# Autodesk Inventor assembly: RightGantryMount
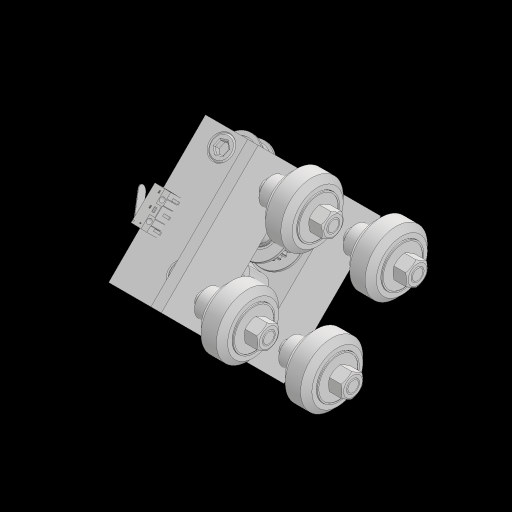
[picture p0: Inventor's stored thumbnail of the model, 512x512]
Saved by Autodesk Inventor 2023 (Build 270158000, 158)
## iProperties
Created: 2023-07-18
Part Number: RightGantryMount
Document SubType Name: Assembly
Designer: tandu
Author: tandu
## Documents named in this file (8)
- C:\Users\tandu\Documents\GrabCAD\Custom Conveyor Belt 3D Printer\References\Roller based conveyor belt 3d printer\RightGantryMount.iam
- C:\Users\tandu\Documents\GrabCAD\Custom Conveyor Belt 3D Printer\References\Roller based conveyor belt 3d printer\RollerVersiongantry_mount_right_bottom_v2.ipt
- C:\Users\tandu\Documents\GrabCAD\Custom Conveyor Belt 3D Printer\References\Roller based conveyor belt 3d printer\RollerVersionGates_2GT_20T_Toothed_Idler_Vychoz¡.ipt
- C:\Users\tandu\Documents\GrabCAD\Custom Conveyor Belt 3D Printer\References\Roller based conveyor belt 3d printer\RollerVersionF695 Bearing.step.ipt
- C:\Users\tandu\Documents\GrabCAD\Custom Conveyor Belt 3D Printer\References\Roller based conveyor belt 3d printer\RollerVersiongantry_mount_right_top_v2.ipt
- C:\Users\tandu\Documents\GrabCAD\Custom Conveyor Belt 3D Printer\References\Roller based conveyor belt 3d printer\RollerVersionM5x40.ipt
- C:\Users\tandu\Documents\GrabCAD\Custom Conveyor Belt 3D Printer\References\Roller based conveyor belt 3d printer\RollerVersionMicroswitch2.step.iam
- C:\Users\tandu\Documents\GrabCAD\Custom Conveyor Belt 3D Printer\References\Roller based conveyor belt 3d printer\RollerVersionSVWB.iam
## Components (13 placed, 7 different names)
1. RollerVersiongantry_mount_right_bottom_v2:1 — Insert:3, Insert:4, Insert:8, Mate:1
2. RollerVersionGates_2GT_20T_Toothed_Idler_Vychoz¡:1 — Insert:7
3. RollerVersionF695 Bearing.step:1 — Insert:6
4. RollerVersionF695 Bearing.step:2 — Insert:5, Insert:6
5. RollerVersiongantry_mount_right_top_v2:1 — Insert:1, Insert:2, Insert:5, Insert:7, Insert:8, Mate:1, Insert:9, Insert:10, Insert:11
6. RollerVersionM5x40:1 — Insert:10
7. RollerVersionM5x40:2 — Insert:9
8. RollerVersionM5x40:3 — Insert:11
9. RollerVersionMicroswitch2.step:1 [sub-assembly]
10. RollerVersionSVWB:1 [sub-assembly] — Insert:2
11. RollerVersionSVWB:2 [sub-assembly] — Insert:4
12. RollerVersionSVWB:3 [sub-assembly] — Insert:3
13. RollerVersionSVWB:4 [sub-assembly] — Insert:1
## Relationships (12: Insert 11, Mate 1)
- Insert:1: RollerVersiongantry_mount_right_top_v2:1 ↔ RollerVersionSVWB:4
- Insert:2: RollerVersiongantry_mount_right_top_v2:1 ↔ RollerVersionSVWB:1
- Insert:3: RollerVersiongantry_mount_right_bottom_v2:1 ↔ RollerVersionSVWB:3
- Insert:4: RollerVersiongantry_mount_right_bottom_v2:1 ↔ RollerVersionSVWB:2
- Insert:5: RollerVersionF695 Bearing.step:2 ↔ RollerVersiongantry_mount_right_top_v2:1
- Insert:6: RollerVersionF695 Bearing.step:1 ↔ RollerVersionF695 Bearing.step:2
- Insert:7: RollerVersionGates_2GT_20T_Toothed_Idler_Vychoz¡:1 ↔ RollerVersiongantry_mount_right_top_v2:1
- Insert:8: RollerVersiongantry_mount_right_bottom_v2:1 ↔ RollerVersiongantry_mount_right_top_v2:1
- Mate:1: RollerVersiongantry_mount_right_bottom_v2:1 ↔ RollerVersiongantry_mount_right_top_v2:1
- Insert:9: RollerVersiongantry_mount_right_top_v2:1 ↔ RollerVersionM5x40:2
- Insert:10: RollerVersiongantry_mount_right_top_v2:1 ↔ RollerVersionM5x40:1
- Insert:11: RollerVersiongantry_mount_right_top_v2:1 ↔ RollerVersionM5x40:3
